# Autodesk Inventor assembly: Montagem1
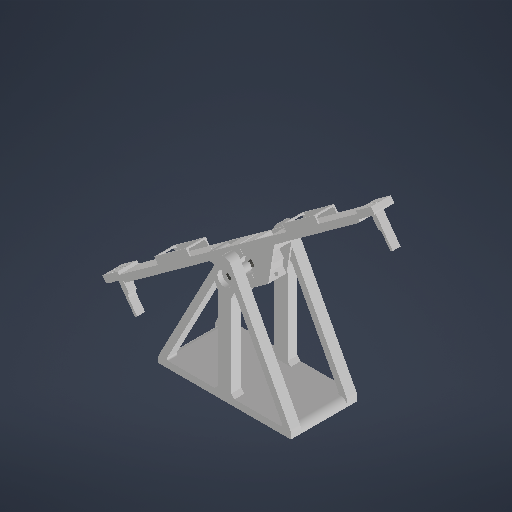
[picture p0: Inventor's stored thumbnail of the model, 512x512]
Saved by Autodesk Inventor 2026 (Build 300175050, 175E)
## iProperties
Created: 2025-03-14
Part Number: Montagem1
Document SubType Name: Assembly
Designer: Ian
Author: Ian
## Documents named in this file (5)
- C:\Users\Ian\Desktop\Drone\BaseTestes\Base de Testes\Projeto\Montagem1.iam
- C:\Users\Ian\Desktop\Drone\BaseTestes\Base de Testes\Projeto\EixoMotores.ipt
- C:\Users\Ian\Desktop\Drone\BaseTestes\Base de Testes\Projeto\Base.ipt
- C:\Users\Ian\Desktop\Drone\BaseTestes\Base de Testes\Projeto\eixoBase.ipt
- C:\Users\Ian\Desktop\Drone\BaseTestes\Base de Testes\Projeto\Espaçadores.ipt
## Components (6 placed, 4 different names)
1. Base:1 — Coincidente:5, Coincidente:6, Alinhado:2, Alinhado:3, Coincidente:13, Coincidente:14, Coincidente:15, Coincidente:16, Alinhado:5
2. eixoBase:1 — Coincidente:6, Coincidente:10, Alinhado:2, Alinhado:3, Coincidente:11, Coincidente:12
3. EixoMotores:1 — Coincidente:7, Coincidente:8, Coincidente:9, Coincidente:10, Coincidente:15, Coincidente:16
4. EixoMotores:2 — Coincidente:7, Coincidente:8, Coincidente:9
5. Espaçadores:1 — Coincidente:12, Coincidente:14
6. Espaçadores:2 — Coincidente:11, Coincidente:13
## Relationships (16: Mate 12, Flush 4)
- Alinhado:1 [Flush]
- Coincidente:5 [Mate]: Base:1
- Coincidente:6 [Mate]: Base:1 ↔ eixoBase:1
- Coincidente:7 [Mate]: EixoMotores:1 ↔ EixoMotores:2
- Coincidente:8 [Mate]: EixoMotores:1 ↔ EixoMotores:2
- Coincidente:9 [Mate]: EixoMotores:1 ↔ EixoMotores:2
- Coincidente:10 [Mate]: eixoBase:1 ↔ EixoMotores:1
- Alinhado:2 [Flush]: Base:1 ↔ eixoBase:1
- Alinhado:3 [Flush]: Base:1 ↔ eixoBase:1
- Coincidente:11 [Mate]: eixoBase:1 ↔ Espaçadores:2
- Coincidente:12 [Mate]: eixoBase:1 ↔ Espaçadores:1
- Coincidente:13 [Mate]: Base:1 ↔ Espaçadores:2
- Coincidente:14 [Mate]: Base:1 ↔ Espaçadores:1
- Coincidente:15 [Mate] (20 mm): Base:1 ↔ EixoMotores:1
- Coincidente:16 [Mate] (20 mm): Base:1 ↔ EixoMotores:1
- Alinhado:5 [Flush]: Base:1
